# Autodesk Inventor assembly: Assembly Servo
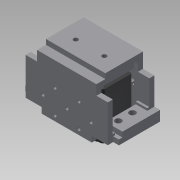
[picture p0: Inventor's stored thumbnail of the model, 180x180]
Saved by Autodesk Inventor 2015 SP1 (Build 190203100, 203)
## iProperties
Created: 2015-03-14
Part Number: Assembly Servo
Document SubType Name: Assembly
Designer: Rafi Kurnia Putra
Author: Rafi Kurnia Putra
## Documents named in this file (4)
- D:\Dropbox\krpai berkaki trui 2015\ROBUSTA\MEKANIK\ROBUSTA\Assembly Servo.iam
- D:\Dropbox\krpai berkaki trui 2015\ROBUSTA\MEKANIK\ROBUSTA\Braket Servo 2.ipt
- D:\Dropbox\krpai berkaki trui 2015\ROBUSTA\MEKANIK\ROBUSTA\servo.ipt
- D:\Dropbox\krpai berkaki trui 2015\ROBUSTA\MEKANIK\ROBUSTA\Bracket3.ipt
## Components (3 placed, 3 different names)
1. Braket Servo 2:1 — Flush:1, Flush:2, Flush:3, Flush:5, Mate:1, Mate:2, Mate:3
2. Bracket3:1 — Flush:5
3. servo:1 — Mate:1, Mate:2, Mate:3
## Relationships (7: Flush 4, Mate 3)
- Flush:1: Braket Servo 2:1
- Flush:2: Braket Servo 2:1
- Flush:3: Braket Servo 2:1
- Flush:5: Braket Servo 2:1 ↔ Bracket3:1
- Mate:1: Braket Servo 2:1 ↔ servo:1
- Mate:2: Braket Servo 2:1 ↔ servo:1
- Mate:3: Braket Servo 2:1 ↔ servo:1
